# Autodesk Inventor assembly: EV-ADF4360
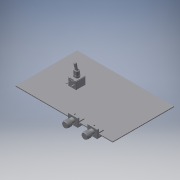
[picture p0: Inventor's stored thumbnail of the model, 180x180]
Saved by Autodesk Inventor 2018 (Build 220112000, 112)
## iProperties
Created: 2018-04-06
Part Number: EV-ADF4360
Document SubType Name: Assembly
Designer: bbramman
Author: bbramman
## Documents named in this file (4)
- C:\Users\bbramman\OneDrive\Documents\Trapped Ion Research (Grad)\Electronics\pll-evalboard-synthesizer\Box CAD\EV-ADF4360.iam
- C:\Users\bbramman\OneDrive\Documents\Trapped Ion Research (Grad)\Electronics\pll-evalboard-synthesizer\Box CAD\95x60mm-PCB.ipt
- C:\Users\bbramman\OneDrive\Documents\Trapped Ion Research (Grad)\Electronics\pll-evalboard-synthesizer\Box CAD\Switch.iam
- C:\Users\bbramman\OneDrive\Documents\Trapped Ion Research (Grad)\Electronics\pll-evalboard-synthesizer\Box CAD\SMA-END.ipt
## Components (4 placed, 3 different names)
1. 95x60mm-PCB:1 — Mate:1, Mate:2, Mate:3, Mate:4, Mate:5, Flush:1, Flush:2
2. Switch:1 [sub-assembly] — Mate:1, Flush:1, Flush:2
3. SMA-END:1 — Mate:2, Mate:5
4. SMA-END:2 — Mate:3, Mate:4
## Relationships (7: Mate 5, Flush 2)
- Mate:1: 95x60mm-PCB:1 ↔ Switch:1
- Mate:2: 95x60mm-PCB:1 ↔ SMA-END:1
- Mate:3: 95x60mm-PCB:1 ↔ SMA-END:2
- Mate:4: 95x60mm-PCB:1 ↔ SMA-END:2
- Mate:5: 95x60mm-PCB:1 ↔ SMA-END:1
- Flush:1 (25.4 mm): 95x60mm-PCB:1 ↔ Switch:1
- Flush:2 (25.4 mm): 95x60mm-PCB:1 ↔ Switch:1
